# Autodesk Inventor assembly: Intake
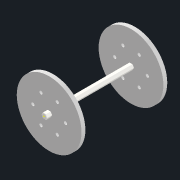
[picture p0: Inventor's stored thumbnail of the model, 180x180]
Saved by Autodesk Inventor 2022 (Build 260153000, 153)
## iProperties
Created: 2021-12-07
Part Number: Intake
Document SubType Name: Assembly
Designer: divid
Author: divid
## Documents named in this file (3)
- C:\Users\divid\Documents\GitHub\ComputerAidedDesign\2021-22\FTC\#13822 Robovikes\Intake\Intake.iam
- C:\Users\divid\Documents\GitHub\ComputerAidedDesign\2021-22\FTC\#13822 Robovikes\Intake\Input _Ring.ipt
- C:\Users\divid\Documents\GitHub\ComputerAidedDesign\2021-22\FTC\#13822 Robovikes\Intake\5mm x 90mm Hex Shaft - 4 Pack.ipt
## Components (3 placed, 2 different names)
1. Input _Ring:1 — Flush:1, Flush:2, Mate:1, Mate:2
2. Input _Ring:2 — Flush:1, Flush:2
3. 5mm x 90mm Hex Shaft - 4 Pack:1 — Mate:1, Mate:2
## Relationships (4: Flush 2, Mate 2)
- Flush:1: Input _Ring:1 ↔ Input _Ring:2
- Flush:2: Input _Ring:1 ↔ Input _Ring:2
- Mate:1: Input _Ring:1 ↔ 5mm x 90mm Hex Shaft - 4 Pack:1
- Mate:2: Input _Ring:1 ↔ 5mm x 90mm Hex Shaft - 4 Pack:1
